# Autodesk Inventor assembly: Subensamble_mesa
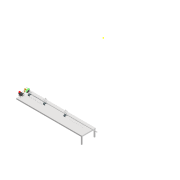
[picture p0: Inventor's stored thumbnail of the model, 180x180]
Saved by Autodesk Inventor 2021 (Build 250183000, 183)
## iProperties
Created: 2021-04-29
Part Number: Subensamble_mesa
Document SubType Name: Assembly
Designer: Admin
Author: Admin
## Documents named in this file (29)
- C:\Users\maaro\Documents\UNAL\Automatización de Procesos de Manufactura\Github\Proyecto_APM\CADs estaciones a automatizar\Estación corte\Subensamble_mesa.iam
- C:\Users\maaro\Documents\UNAL\Automatización de Procesos de Manufactura\Github\Proyecto_APM\CADs estaciones a automatizar\Estación corte\Mesa_cortadora.ipt
- C:\Users\maaro\Documents\UNAL\Automatización de Procesos de Manufactura\Github\Proyecto_APM\CADs estaciones a automatizar\Estación corte\Pata_mesa.ipt
- C:\Users\maaro\Documents\UNAL\Automatización de Procesos de Manufactura\Github\Proyecto_APM\CADs estaciones a automatizar\Estación corte\Tubo-2_1_8.ipt
- C:\Users\maaro\Documents\UNAL\Automatización de Procesos de Manufactura\Github\Proyecto_APM\CADs estaciones a automatizar\Estación corte\Base soporte tubos.ipt
- C:\Users\maaro\Documents\UNAL\Automatización de Procesos de Manufactura\Github\Proyecto_APM\CADs estaciones a automatizar\Estación corte\193992 DSNU-32-60-PPS-A---(60PPSA---00--0-------0).iam
- C:\Users\maaro\Documents\UNAL\Automatización de Procesos de Manufactura\Github\Proyecto_APM\CADs estaciones a automatizar\Estación corte\Eje roscado base soporte tubo.ipt
- C:\Users\maaro\Documents\UNAL\Automatización de Procesos de Manufactura\Github\Proyecto_APM\CADs estaciones a automatizar\Estación corte\Soporte Superior Tubos.ipt
- C:\Users\maaro\Documents\UNAL\Automatización de Procesos de Manufactura\Github\Proyecto_APM\CADs estaciones a automatizar\Estación corte\Soporte Pistón.ipt
- C:\Users\maaro\Documents\Inventor\Content Center Files\R2021\en-US\ISO 4035(2)\ISO 4035 - M16 - ISO.ipt
- C:\Users\maaro\Documents\UNAL\Automatización de Procesos de Manufactura\Github\Proyecto_APM\CADs estaciones a automatizar\Estación corte\Eje roscado base soporte tubo_MIR.ipt
- C:\Users\maaro\Documents\UNAL\Automatización de Procesos de Manufactura\Github\Proyecto_APM\CADs estaciones a automatizar\Estación corte\193992 DSNU-32-60-PPS-A---(60PPSA---00--0-------0)_MIR.iam
- C:\Users\maaro\Documents\UNAL\Automatización de Procesos de Manufactura\Github\Proyecto_APM\CADs estaciones a automatizar\Estación corte\Base soporte tubos_MIR.ipt
- C:\Users\maaro\Documents\UNAL\Automatización de Procesos de Manufactura\Github\Proyecto_APM\CADs estaciones a automatizar\Estación corte\Eje roscado base soporte tubo_MIR1.ipt
- C:\Users\maaro\Documents\UNAL\Automatización de Procesos de Manufactura\Github\Proyecto_APM\CADs estaciones a automatizar\Estación corte\Soporte Superior Tubos_MIR.ipt
- C:\Users\maaro\Documents\UNAL\Automatización de Procesos de Manufactura\Github\Proyecto_APM\CADs estaciones a automatizar\Estación corte\Soporte Pistón_MIR.ipt
- C:\Users\maaro\Documents\UNAL\Automatización de Procesos de Manufactura\Github\Proyecto_APM\CADs estaciones a automatizar\Estación corte\Eje roscado base soporte tubo_MIR_MIR.ipt
- C:\Users\maaro\Documents\UNAL\Automatización de Procesos de Manufactura\Github\Proyecto_APM\CADs estaciones a automatizar\Estación corte\Subensamble_cortadora_MIR.iam
- C:\Users\maaro\Documents\UNAL\Automatización de Procesos de Manufactura\Github\Proyecto_APM\CADs estaciones a automatizar\Estación corte\PerfilZ.ipt
- C:\Users\maaro\Documents\UNAL\Automatización de Procesos de Manufactura\Github\Proyecto_APM\CADs estaciones a automatizar\Estación corte\V-Groove_Roller.ipt
- C:\Users\maaro\Documents\UNAL\Automatización de Procesos de Manufactura\Github\Proyecto_APM\CADs estaciones a automatizar\Estación corte\Base soporte tubos MOVIL.ipt
- C:\Users\maaro\Documents\UNAL\Automatización de Procesos de Manufactura\Github\Proyecto_APM\CADs estaciones a automatizar\Estación corte\Angulo en V.ipt
- C:\Users\maaro\Documents\Inventor\Content Center Files\R2021\en-US\ISO 7050 - F-H(1)\DIN EN ISO 7050 - ST6,3 x 25 - F - H.ipt
- C:\Users\maaro\Documents\Inventor\Content Center Files\R2021\en-US\DIN EN ISO 4032\DIN EN ISO 4032 - M6.ipt
- C:\Users\maaro\Documents\UNAL\Automatización de Procesos de Manufactura\Github\Proyecto_APM\CADs estaciones a automatizar\Estación corte\PerfilZ_MIR.ipt
- C:\Users\maaro\Documents\UNAL\Automatización de Procesos de Manufactura\Github\Proyecto_APM\CADs estaciones a automatizar\Estación corte\V-Groove_Roller_MIR.ipt
- C:\Users\maaro\Documents\UNAL\Automatización de Procesos de Manufactura\Github\Proyecto_APM\CADs estaciones a automatizar\Estación corte\Angulo en V_MIR.ipt
- C:\Users\maaro\Documents\UNAL\Automatización de Procesos de Manufactura\Github\Proyecto_APM\CADs estaciones a automatizar\Estación corte\Agarre Cortadora.ipt
- C:\Users\maaro\Documents\UNAL\Automatización de Procesos de Manufactura\Github\Proyecto_APM\CADs estaciones a automatizar\Estación corte\AIS2021\CP96SDB40-160-M9PM(160_0_0).iam
## Components (60 placed, 28 different names)
1. Mesa_cortadora:1 — Coincidencia:1, Coincidencia:2, Coincidencia:3, Coincidencia:4, Coincidencia:5, Coincidencia:6, Coincidencia:7, Coincidencia:8, Coincidencia:9, Coincidencia:10, Coincidencia:11, Coincidencia:12, Mate:15, Flush:1, Flush:2, Flush:3, Mate:80, Flush:17, Mate:83, Mate:84, Mate:85, Flush:18, Mate:89, Flush:20
2. Pata_mesa:1 — Coincidencia:7, Coincidencia:8, Coincidencia:9
3. Pata_mesa:2 — Coincidencia:1, Coincidencia:2, Coincidencia:3
4. Pata_mesa:3 — Coincidencia:4, Coincidencia:5, Coincidencia:6
5. Pata_mesa:4 — Coincidencia:10, Coincidencia:11, Coincidencia:12
6. Tubo-2_1_8:1 — Tangent:1, Tangent:2, Flush:7
7. Base soporte tubos:1 — Mate:15, Tangent:1, Tangent:2, Flush:1, Flush:2
8. 193992 DSNU-32-60-PPS-A---(60PPSA---00--0-------0):2 [sub-assembly] — Mate:18, Flush:10, Flush:11
9. Base soporte tubos MOVIL:1 — Flush:3, Flush:5, Flush:6, Flush:8, Flush:9, Mate:23, Mate:25, Mate:31, Mate:36, Mate:37, Mate:38, Flush:12, Mate:89, Mate:90
10. Eje roscado base soporte tubo:1 — Flush:5, Flush:6, Mate:20, Mate:22, Mate:24, Mate:26, Mate:31, Mate:32, Mate:33
11. Soporte Superior Tubos:1 — Flush:7, Flush:8, Flush:9, Mate:18, Symmetry:1, Mate:33
12. Soporte Pistón:1 — Flush:10, Flush:11, Mate:19, Mate:21, Symmetry:1, Mate:32, Mate:34, Mate:35, Flush:13, Mate:39
13. ISO 4035 M16:1 — Mate:21, Mate:22
14. ISO 4035 M16:2 — Mate:19, Mate:20
15. ISO 4035 M16:3 — Mate:23, Mate:24
16. ISO 4035 M16:4 — Mate:25, Mate:26
17. Eje roscado base soporte tubo_MIR:1 — Mate:27, Mate:28, Mate:29, Mate:30, Mate:38, Flush:12, Flush:13, Mate:39
18. ISO 4035 M16:5 — Mate:27, Mate:34
19. ISO 4035 M16:6 — Mate:28, Mate:35
20. ISO 4035 M16:7 — Mate:29, Mate:37
21. ISO 4035 M16:8 — Mate:30, Mate:36
22. 193992 DSNU-32-60-PPS-A---(60PPSA---00--0-------0)_MIR:1 [sub-assembly] — Mate:44, Mate:48, Mate:49
23. Base soporte tubos_MIR:1 — Mate:40, Mate:41, Mate:42, Mate:45, Mate:46, Mate:55, Mate:57, Flush:16, Mate:59, Mate:64, Mate:66, Mate:72, Mate:74, Mate:76, Mate:78, Mate:80, Flush:17
24. Eje roscado base soporte tubo_MIR1:1 — Mate:40, Mate:41, Mate:42, Mate:43, Mate:47, Mate:50, Mate:52, Mate:73, Mate:77
25. Soporte Superior Tubos_MIR:1 — Mate:43, Mate:44, Mate:45, Mate:46, Symmetry:2
26. Soporte Pistón_MIR:1 — Mate:47, Mate:48, Mate:49, Symmetry:2, Mate:58, Flush:15, Mate:62, Mate:69, Mate:71, Mate:81, Mate:82
27. ISO 4035 M16:9 — Mate:50, Mate:82
28. ISO 4035 M16:10 — Mate:52, Mate:71
29. ISO 4035 M16:11 — Mate:55, Mate:76, Mate:77
30. ISO 4035 M16:12 — Mate:57, Mate:72, Mate:73
31. Eje roscado base soporte tubo_MIR_MIR:1 — Mate:58, Flush:15, Flush:16, Mate:59, Mate:61, Mate:70, Mate:75, Mate:79
32. ISO 4035 M16:13 — Mate:61, Mate:81
33. ISO 4035 M16:14 — Mate:62, Mate:69, Mate:70
34. ISO 4035 M16:15 — Mate:64, Mate:78, Mate:79
35. ISO 4035 M16:16 — Mate:66, Mate:74, Mate:75
36. Subensamble_cortadora_MIR:1 [sub-assembly] — Mate:83, Flush:22, Mate:94
37. PerfilZ:2 — Mate:84, Mate:85, Flush:18, Flush:19, Mate:86, Mate:87, Mate:88
38. V-Groove_Roller:1 — Tangent:3, Tangent:4, Insert:1, Insert:2, Insert:3, Insert:4
39. Angulo en V:1 — Flush:19, Mate:86, Mate:87, Mate:88, Tangent:3, Tangent:4
40. DIN EN ISO 4032 M6:1 — Insert:1
41. DIN EN ISO 4032 M6:2 — Insert:2
42. DIN EN ISO 4032 M6:3 — Insert:3
43. DIN EN ISO 4032 M6:4 — Insert:4
44. PerfilZ_MIR:1 — Mate:91, Mate:92, Mate:93, Flush:21
45. V-Groove_Roller_MIR:1 — Tangent:5, Tangent:6, Insert:5, Insert:6, Insert:7, Insert:8
46. Angulo en V_MIR:1 — Tangent:5, Tangent:6, Mate:91, Mate:92, Mate:93, Flush:21
47. DIN EN ISO 4032 M6:5 — Insert:5
48. DIN EN ISO 4032 M6:6 — Insert:6
49. DIN EN ISO 4032 M6:7 — Insert:7
50. DIN EN ISO 4032 M6:8 — Insert:8
51. DIN EN ISO 7050 - F-H ST6,3 x 25 - F - H:5
52. DIN EN ISO 7050 - F-H ST6,3 x 25 - F - H:6
53. DIN EN ISO 7050 - F-H ST6,3 x 25 - F - H:7
54. DIN EN ISO 7050 - F-H ST6,3 x 25 - F - H:8
55. Agarre Cortadora:1 — Flush:23, Flush:24, Mate:94
56. CP96SDB40-160-M9PM(160_0_0):1 [sub-assembly]
57. DIN EN ISO 7050 - F-H ST6,3 x 25 - F - H:1 — Mate:90
58. DIN EN ISO 7050 - F-H ST6,3 x 25 - F - H:2
59. DIN EN ISO 7050 - F-H ST6,3 x 25 - F - H:3
60. DIN EN ISO 7050 - F-H ST6,3 x 25 - F - H:4
## Component patterns: (4 elements, first: DIN EN ISO 7050 - F-H ST6,3 x 25 - F - H:1)
## Relationships (119: Mate 81, Flush 22, Insert 8, Tangent 6, Symmetry 2)
- Coincidencia:1 [Mate]: Mesa_cortadora:1 ↔ Pata_mesa:2
- Coincidencia:2 [Mate]: Mesa_cortadora:1 ↔ Pata_mesa:2
- Coincidencia:3 [Mate]: Mesa_cortadora:1 ↔ Pata_mesa:2
- Coincidencia:4 [Mate]: Mesa_cortadora:1 ↔ Pata_mesa:3
- Coincidencia:5 [Mate]: Mesa_cortadora:1 ↔ Pata_mesa:3
- Coincidencia:6 [Mate]: Mesa_cortadora:1 ↔ Pata_mesa:3
- Coincidencia:7 [Mate]: Mesa_cortadora:1 ↔ Pata_mesa:1
- Coincidencia:8 [Mate]: Mesa_cortadora:1 ↔ Pata_mesa:1
- Coincidencia:9 [Mate]: Mesa_cortadora:1 ↔ Pata_mesa:1
- Coincidencia:10 [Mate]: Mesa_cortadora:1 ↔ Pata_mesa:4
- Coincidencia:11 [Mate]: Mesa_cortadora:1 ↔ Pata_mesa:4
- Coincidencia:12 [Mate]: Mesa_cortadora:1 ↔ Pata_mesa:4
- Mate:15: Mesa_cortadora:1 ↔ Base soporte tubos:1
- Tangent:1: Tubo-2_1_8:1 ↔ Base soporte tubos:1
- Tangent:2: Tubo-2_1_8:1 ↔ Base soporte tubos:1
- Flush:1 (297.3 mm): Mesa_cortadora:1 ↔ Base soporte tubos:1
- Flush:2 (1220 mm): Mesa_cortadora:1 ↔ Base soporte tubos:1
- Flush:3 (297 mm): Mesa_cortadora:1 ↔ Base soporte tubos MOVIL:1
- Flush:5: Base soporte tubos MOVIL:1 ↔ Eje roscado base soporte tubo:1
- Flush:6 (20 mm): Base soporte tubos MOVIL:1 ↔ Eje roscado base soporte tubo:1
- Flush:7: Tubo-2_1_8:1 ↔ Soporte Superior Tubos:1
- Flush:8: Base soporte tubos MOVIL:1 ↔ Soporte Superior Tubos:1
- Flush:9: Base soporte tubos MOVIL:1 ↔ Soporte Superior Tubos:1
- Mate:18: 193992 DSNU-32-60-PPS-A---(60PPSA---00--0-------0):2 ↔ Soporte Superior Tubos:1
- Flush:10: 193992 DSNU-32-60-PPS-A---(60PPSA---00--0-------0):2 ↔ Soporte Pistón:1
- Flush:11: 193992 DSNU-32-60-PPS-A---(60PPSA---00--0-------0):2 ↔ Soporte Pistón:1
- Mate:19: Soporte Pistón:1 ↔ ISO 4035 M16:2
- Mate:20: Eje roscado base soporte tubo:1 ↔ ISO 4035 M16:2
- Mate:21: Soporte Pistón:1 ↔ ISO 4035 M16:1
- Mate:22: Eje roscado base soporte tubo:1 ↔ ISO 4035 M16:1
- Mate:23: Base soporte tubos MOVIL:1 ↔ ISO 4035 M16:3
- Mate:24: Eje roscado base soporte tubo:1 ↔ ISO 4035 M16:3
- Mate:25: Base soporte tubos MOVIL:1 ↔ ISO 4035 M16:4
- Mate:26: Eje roscado base soporte tubo:1 ↔ ISO 4035 M16:4
- Symmetry:1: Soporte Superior Tubos:1 ↔ Soporte Pistón:1
- Mate:27: Eje roscado base soporte tubo_MIR:1 ↔ ISO 4035 M16:5
- Mate:28: Eje roscado base soporte tubo_MIR:1 ↔ ISO 4035 M16:6
- Mate:29: Eje roscado base soporte tubo_MIR:1 ↔ ISO 4035 M16:7
- Mate:30: Eje roscado base soporte tubo_MIR:1 ↔ ISO 4035 M16:8
- Mate:31: Base soporte tubos MOVIL:1 ↔ Eje roscado base soporte tubo:1
- Mate:32: Eje roscado base soporte tubo:1 ↔ Soporte Pistón:1
- Mate:33: Eje roscado base soporte tubo:1 ↔ Soporte Superior Tubos:1
- Mate:34: Soporte Pistón:1 ↔ ISO 4035 M16:5
- Mate:35: Soporte Pistón:1 ↔ ISO 4035 M16:6
- Mate:36: Base soporte tubos MOVIL:1 ↔ ISO 4035 M16:8
- Mate:37: Base soporte tubos MOVIL:1 ↔ ISO 4035 M16:7
- Mate:38: Base soporte tubos MOVIL:1 ↔ Eje roscado base soporte tubo_MIR:1
- Flush:12 (-20 mm): Base soporte tubos MOVIL:1 ↔ Eje roscado base soporte tubo_MIR:1
- Flush:13 (-27.5 mm): Soporte Pistón:1 ↔ Eje roscado base soporte tubo_MIR:1
- Mate:39: Soporte Pistón:1 ↔ Eje roscado base soporte tubo_MIR:1
- Mate:40: Base soporte tubos_MIR:1 ↔ Eje roscado base soporte tubo_MIR1:1
- Mate:41 (20 mm): Base soporte tubos_MIR:1 ↔ Eje roscado base soporte tubo_MIR1:1
- Mate:42: Base soporte tubos_MIR:1 ↔ Eje roscado base soporte tubo_MIR1:1
- Mate:43: Eje roscado base soporte tubo_MIR1:1 ↔ Soporte Superior Tubos_MIR:1
- Mate:44: 193992 DSNU-32-60-PPS-A---(60PPSA---00--0-------0)_MIR:1 ↔ Soporte Superior Tubos_MIR:1
- Mate:45: Base soporte tubos_MIR:1 ↔ Soporte Superior Tubos_MIR:1
- Mate:46: Base soporte tubos_MIR:1 ↔ Soporte Superior Tubos_MIR:1
- Mate:47: Eje roscado base soporte tubo_MIR1:1 ↔ Soporte Pistón_MIR:1
- Mate:48: 193992 DSNU-32-60-PPS-A---(60PPSA---00--0-------0)_MIR:1 ↔ Soporte Pistón_MIR:1
- Mate:49: 193992 DSNU-32-60-PPS-A---(60PPSA---00--0-------0)_MIR:1 ↔ Soporte Pistón_MIR:1
- Mate:50: Eje roscado base soporte tubo_MIR1:1 ↔ ISO 4035 M16:9
- Mate:52: Eje roscado base soporte tubo_MIR1:1 ↔ ISO 4035 M16:10
- Mate:55: Base soporte tubos_MIR:1 ↔ ISO 4035 M16:11
- Mate:57: Base soporte tubos_MIR:1 ↔ ISO 4035 M16:12
- Symmetry:2: Soporte Superior Tubos_MIR:1 ↔ Soporte Pistón_MIR:1
- Mate:58: Soporte Pistón_MIR:1 ↔ Eje roscado base soporte tubo_MIR_MIR:1
- Flush:15 (-27.5 mm): Soporte Pistón_MIR:1 ↔ Eje roscado base soporte tubo_MIR_MIR:1
- Flush:16 (-20 mm): Base soporte tubos_MIR:1 ↔ Eje roscado base soporte tubo_MIR_MIR:1
- Mate:59: Base soporte tubos_MIR:1 ↔ Eje roscado base soporte tubo_MIR_MIR:1
- Mate:61: Eje roscado base soporte tubo_MIR_MIR:1 ↔ ISO 4035 M16:13
- Mate:62: Soporte Pistón_MIR:1 ↔ ISO 4035 M16:14
- Mate:64: Base soporte tubos_MIR:1 ↔ ISO 4035 M16:15
- Mate:66: Base soporte tubos_MIR:1 ↔ ISO 4035 M16:16
- Mate:69: Soporte Pistón_MIR:1 ↔ ISO 4035 M16:14
- Mate:70: Eje roscado base soporte tubo_MIR_MIR:1 ↔ ISO 4035 M16:14
- Mate:71: Soporte Pistón_MIR:1 ↔ ISO 4035 M16:10
- Mate:72: Base soporte tubos_MIR:1 ↔ ISO 4035 M16:12
- Mate:73: Eje roscado base soporte tubo_MIR1:1 ↔ ISO 4035 M16:12
- Mate:74: Base soporte tubos_MIR:1 ↔ ISO 4035 M16:16
- Mate:75: Eje roscado base soporte tubo_MIR_MIR:1 ↔ ISO 4035 M16:16
- Mate:76: Base soporte tubos_MIR:1 ↔ ISO 4035 M16:11
- Mate:77: Eje roscado base soporte tubo_MIR1:1 ↔ ISO 4035 M16:11
- Mate:78: Base soporte tubos_MIR:1 ↔ ISO 4035 M16:15
- Mate:79: Eje roscado base soporte tubo_MIR_MIR:1 ↔ ISO 4035 M16:15
- Mate:80: Mesa_cortadora:1 ↔ Base soporte tubos_MIR:1
- Mate:81: Soporte Pistón_MIR:1 ↔ ISO 4035 M16:13
- Mate:82: Soporte Pistón_MIR:1 ↔ ISO 4035 M16:9
- Flush:17 (297 mm): Mesa_cortadora:1 ↔ Base soporte tubos_MIR:1
- Mate:83: Mesa_cortadora:1 ↔ Subensamble_cortadora_MIR:1
- Mate:84: Mesa_cortadora:1 ↔ PerfilZ:2
- Mate:85: Mesa_cortadora:1 ↔ PerfilZ:2
- Flush:18: Mesa_cortadora:1 ↔ PerfilZ:2
- Flush:19: PerfilZ:2 ↔ Angulo en V:1
- Mate:86: PerfilZ:2 ↔ Angulo en V:1
- Mate:87: PerfilZ:2 ↔ Angulo en V:1
- Mate:88 (4 mm): PerfilZ:2 ↔ Angulo en V:1
- Tangent:3: V-Groove_Roller:1 ↔ Angulo en V:1
- Tangent:4: V-Groove_Roller:1 ↔ Angulo en V:1
- Mate:89 (80 mm): Mesa_cortadora:1 ↔ Base soporte tubos MOVIL:1
- Mate:90: Base soporte tubos MOVIL:1 ↔ DIN EN ISO 7050 - F-H ST6,3 x 25 - F - H:1
- Insert:1: V-Groove_Roller:1 ↔ DIN EN ISO 4032 M6:1
- Insert:2: V-Groove_Roller:1 ↔ DIN EN ISO 4032 M6:2
- Insert:3: V-Groove_Roller:1 ↔ DIN EN ISO 4032 M6:3
- Insert:4: V-Groove_Roller:1 ↔ DIN EN ISO 4032 M6:4
- Flush:20 (-100 mm): Mesa_cortadora:1
- Tangent:5: V-Groove_Roller_MIR:1 ↔ Angulo en V_MIR:1
- Tangent:6: V-Groove_Roller_MIR:1 ↔ Angulo en V_MIR:1
- Mate:91 (4 mm): PerfilZ_MIR:1 ↔ Angulo en V_MIR:1
- Mate:92: PerfilZ_MIR:1 ↔ Angulo en V_MIR:1
- Mate:93: PerfilZ_MIR:1 ↔ Angulo en V_MIR:1
- Flush:21: PerfilZ_MIR:1 ↔ Angulo en V_MIR:1
- Insert:5: V-Groove_Roller_MIR:1 ↔ DIN EN ISO 4032 M6:5
- Insert:6: V-Groove_Roller_MIR:1 ↔ DIN EN ISO 4032 M6:6
- Insert:7: V-Groove_Roller_MIR:1 ↔ DIN EN ISO 4032 M6:7
- Insert:8: V-Groove_Roller_MIR:1 ↔ DIN EN ISO 4032 M6:8
- Flush:22 (-116 mm): Subensamble_cortadora_MIR:1
- Flush:23: Agarre Cortadora:1
- Flush:24: Agarre Cortadora:1
- Mate:94: Subensamble_cortadora_MIR:1 ↔ Agarre Cortadora:1
